# Autodesk Inventor assembly: NewVatAssem
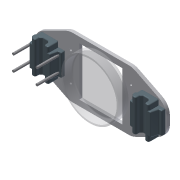
[picture p0: Inventor's stored thumbnail of the model, 180x180]
Saved by Autodesk Inventor 2014 (Build 180170000, 170)
## iProperties
Created: 2015-01-19
Part Number: NewVatAssem
Document SubType Name: Assembly
Designer: Peele
Author: Peele
## Documents named in this file (5)
- E:\Copy\DLP\DMP-SL-v2\SubAssem\NewVatAssem.iam
- E:\Copy\DLP\DMP-SL-v2\CustomParts\VatPlate.ipt
- E:\Copy\DLP\DMP-SL-v2\StockParts\bLOCK.ipt
- E:\Copy\DLP\DMP-SL-v2\StockParts\Petri.ipt
- E:\Copy\DLP\DMP-SL-v2\StockParts\4mmScrew.ipt
## Components (8 placed, 4 different names)
1. VatPlate:1 — Mate:1, Mate:2, Mate:3, Mate:4, Mate:5, Mate:6, Mate:7, Flush:2, Mate:8, Mate:9, Mate:11, Mate:12, Mate:13, Mate:14, Mate:15
2. bLOCK:1 — Mate:1, Mate:2, Mate:3
3. bLOCK:2 — Mate:4, Mate:5, Mate:6
4. Petri:1 — Mate:9, Mate:10, Flush:3
5. 4mmScrew:1 — Mate:11, Flush:4, Flush:5, Mate:12
6. 4mmScrew:2 — Flush:4, Mate:13
7. 4mmScrew:3 — Flush:5, Flush:6, Mate:15
8. 4mmScrew:4 — Flush:6, Mate:14
## Relationships (20: Mate 15, Flush 5)
- Mate:1: VatPlate:1 ↔ bLOCK:1
- Mate:2: VatPlate:1 ↔ bLOCK:1
- Mate:3: VatPlate:1 ↔ bLOCK:1
- Mate:4: VatPlate:1 ↔ bLOCK:2
- Mate:5: VatPlate:1 ↔ bLOCK:2
- Mate:6: VatPlate:1 ↔ bLOCK:2
- Mate:7: VatPlate:1
- Flush:2: VatPlate:1
- Mate:8: VatPlate:1
- Mate:9: VatPlate:1 ↔ Petri:1
- Mate:10: Petri:1
- Flush:3: Petri:1
- Mate:11: VatPlate:1 ↔ 4mmScrew:1
- Flush:4: 4mmScrew:1 ↔ 4mmScrew:2
- Flush:5: 4mmScrew:1 ↔ 4mmScrew:3
- Flush:6: 4mmScrew:3 ↔ 4mmScrew:4
- Mate:12: VatPlate:1 ↔ 4mmScrew:1
- Mate:13: VatPlate:1 ↔ 4mmScrew:2
- Mate:14: VatPlate:1 ↔ 4mmScrew:4
- Mate:15: VatPlate:1 ↔ 4mmScrew:3
